# Autodesk Inventor assembly: Nozzle
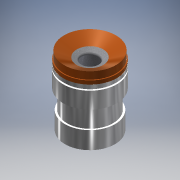
[picture p0: Inventor's stored thumbnail of the model, 180x180]
Saved by Autodesk Inventor 2017 SP1 (Build 210196100, 196)
## iProperties
Created: 2016-10-21
Part Number: Nozzle
Document SubType Name: Assembly
Designer: cflannery
Author: cflannery
## Documents named in this file (7)
- D:\Triton_Rocket_Club\Propulsion\Launches\8-inch-flight\Design\CAD\Nozzle\trunk\Nozzle.iam
- D:\Triton_Rocket_Club\Propulsion\Launches\8-inch-flight\Design\CAD\Nozzle\trunk\aluminum_carrier.ipt
- D:\Triton_Rocket_Club\Propulsion\Launches\8-inch-flight\Design\CAD\Nozzle\trunk\aluminum_retainer.ipt
- D:\Triton_Rocket_Club\Propulsion\Launches\8-inch-flight\Design\CAD\Nozzle\trunk\aluminum_skirt.ipt
- D:\Triton_Rocket_Club\Propulsion\Launches\8-inch-flight\Design\CAD\Nozzle\trunk\graphite.ipt
- D:\Triton_Rocket_Club\Propulsion\Launches\8-inch-flight\Design\CAD\Nozzle\trunk\phenolic_cap.ipt
- D:\Triton_Rocket_Club\Propulsion\Launches\8-inch-flight\Design\CAD\Nozzle\trunk\phenolic_carrier.ipt
## Components (6 placed, 6 different names)
1. aluminum_carrier:1 — Mate:5, Mate:8, Mate:9, Mate:10
2. aluminum_retainer:1 — Mate:4, Mate:9
3. aluminum_skirt:1 — Mate:3, Mate:10
4. graphite:1 — Mate:1, Mate:2, Mate:3, Mate:4, Mate:5, Mate:6, Mate:7
5. phenolic_cap:1 — Mate:1, Mate:6, Mate:8
6. phenolic_carrier:1 — Mate:2, Mate:7
## Relationships (10: Mate 10)
- Mate:1: graphite:1 ↔ phenolic_cap:1
- Mate:2: graphite:1 ↔ phenolic_carrier:1
- Mate:3: aluminum_skirt:1 ↔ graphite:1
- Mate:4: aluminum_retainer:1 ↔ graphite:1
- Mate:5: aluminum_carrier:1 ↔ graphite:1
- Mate:6: graphite:1 ↔ phenolic_cap:1
- Mate:7: graphite:1 ↔ phenolic_carrier:1
- Mate:8: aluminum_carrier:1 ↔ phenolic_cap:1
- Mate:9: aluminum_carrier:1 ↔ aluminum_retainer:1
- Mate:10: aluminum_carrier:1 ↔ aluminum_skirt:1
